# Autodesk Inventor assembly: VersaPlanetaryWithCim
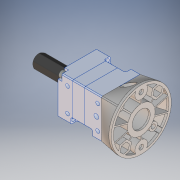
[picture p0: Inventor's stored thumbnail of the model, 180x180]
Saved by Autodesk Inventor 2016 (Build 200138000, 138)
## iProperties
Created: 2016-01-25
Part Number: VersaPlanetaryWithCim
Document SubType Name: Assembly
Designer: CAD
Author: CAD
## Documents named in this file (4)
- C:\Users\PrashantBIA\Desktop\Robotics\Robot Assembly 1-27-15 New Swami\Robot Assembly\Shooter\VersaPlanetaryWithCim.iam
- C:\Users\PrashantBIA\Desktop\Robotics\Robot Assembly 1-27-15 New Swami\Robot Assembly\Shooter\Imported Components\217-4018-STEP-20140806\217-4018-STEP-20140806.ipt
- C:\Users\PrashantBIA\Desktop\Robotics\Robot Assembly 1-27-15 New Swami\Robot Assembly\Shooter\Imported Components\VersaPlanetary-1-Stage-with-BAG-Motor\VersaPlanetary-1-Stage-with-BAG-Motor.iam
- C:\Users\PrashantBIA\Desktop\Robotics\Robot Assembly 1-27-15 New Swami\Robot Assembly\Shooter\miniCIM.ipt
## Components (3 placed, 3 different names)
1. 217-4018-STEP-20140806:1 — Mate:3, Mate:4, Mate:5, Insert:1
2. VersaPlanetary-1-Stage-with-BAG-Motor:1 [sub-assembly] — Mate:3, Mate:4, Mate:5
3. miniCIM:1 — Insert:1
## Relationships (4: Mate 3, Insert 1)
- Mate:3: 217-4018-STEP-20140806:1 ↔ VersaPlanetary-1-Stage-with-BAG-Motor:1
- Mate:4: 217-4018-STEP-20140806:1 ↔ VersaPlanetary-1-Stage-with-BAG-Motor:1
- Mate:5: 217-4018-STEP-20140806:1 ↔ VersaPlanetary-1-Stage-with-BAG-Motor:1
- Insert:1: 217-4018-STEP-20140806:1 ↔ miniCIM:1
